# Autodesk Inventor assembly: Shock
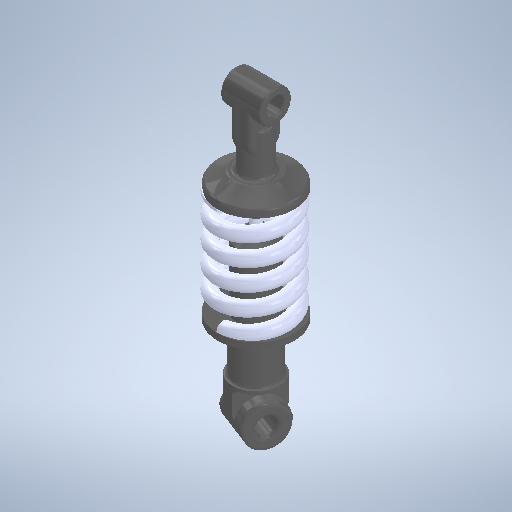
[picture p0: Inventor's stored thumbnail of the model, 512x512]
Saved by Autodesk Inventor 2025 (Build 290162000, 162)
## iProperties
Created: 2022-12-29
Part Number: Shock
Document SubType Name: Assembly
Designer: 5014070
Author: 5014070
Sending System: SolidWorks 2023
Last Author: attic
Last Saved: 2024-12-05
## Documents named in this file (5)
- C:\Users\5014070\Documents\GitHub\Mechanical\SeattleSolarCar2024-2025\Suspension\Front\Cheesed\Shock\Shock.iam
- C:\Users\5014070\Documents\GitHub\Mechanical\SeattleSolarCar2024-2025\Suspension\Front\Cheesed\Shock\Shock Anchor_11.ipt
- C:\Users\5014070\Documents\GitHub\Mechanical\SeattleSolarCar2024-2025\Suspension\Front\Cheesed\Shock\Shock Tube 1_11.ipt
- C:\Users\5014070\Documents\GitHub\Mechanical\SeattleSolarCar2024-2025\Suspension\Front\Cheesed\Shock\Shock Absorber Rod_11.ipt
- C:\Users\5014070\Documents\GitHub\Mechanical\SeattleSolarCar2024-2025\Suspension\Front\Cheesed\Shock\Shock Spring_11.ipt
## Components (4 placed, 4 different names)
1. Shock Anchor_11:1 — Mate:1, Mate:3, Mate:4
2. Shock Tube 1_11:1 — Mate:2, Mate:5, Mate:6
3. Shock Absorber Rod_11:1 — Mate:1, Mate:2, Mate:3
4. Shock Spring_11:1 — Mate:4, Mate:5, Mate:6
## Relationships (6: Mate 6)
- Mate:1: Shock Anchor_11:1 ↔ Shock Absorber Rod_11:1
- Mate:2: Shock Tube 1_11:1 ↔ Shock Absorber Rod_11:1
- Mate:3: Shock Anchor_11:1 ↔ Shock Absorber Rod_11:1
- Mate:4: Shock Anchor_11:1 ↔ Shock Spring_11:1
- Mate:5: Shock Tube 1_11:1 ↔ Shock Spring_11:1
- Mate:6: Shock Tube 1_11:1 ↔ Shock Spring_11:1
